# Autodesk Inventor assembly: 3.000 30A .500 With Adapters
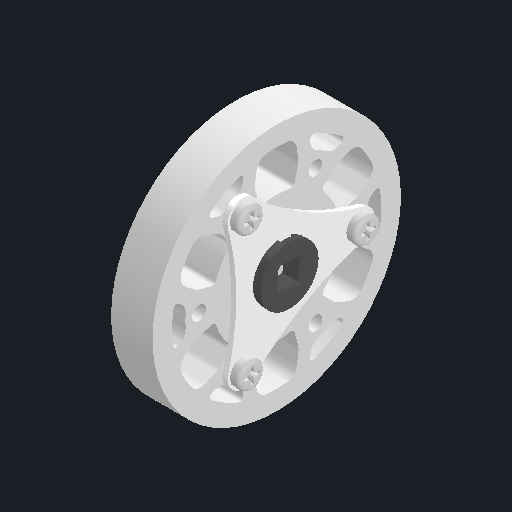
[picture p0: Inventor's stored thumbnail of the model, 512x512]
Saved by Autodesk Inventor 2025 (Build 290162000, 162)
## iProperties
Created: 2024-12-29
Part Number: 3.000 30A .500 With Adapters
Document SubType Name: Assembly
Designer: Averey Ku
Author: Averey Ku
## Documents named in this file (8)
- D:\VEX\High Stakes\CAD\ROBOPROS-CAD-Inventor\Quick Assemblies\3.000 30A .500 With Adapters.iam
- D:\VEX\High Stakes\CAD\ROBOPROS-CAD-Inventor\Motion\Wheels\Flex Wheels\3.000 Flex Wheel\3.000 30A .500.ipt
- D:\VEX\High Stakes\CAD\ROBOPROS-CAD-Inventor\Motion\Wheels\Flex Wheels\3.000 Flex Wheel.ipt
- D:\VEX\High Stakes\CAD\V4\Conveyer\Custom Parts\3 in Flex Wheel Hub.ipt
- D:\VEX\High Stakes\CAD\ROBOPROS-CAD-Inventor\Structure\Standoff\Standoff .50.ipt
- D:\VEX\High Stakes\CAD\ROBOPROS-CAD-Inventor\Structure\Standoff.ipt
- D:\VEX\High Stakes\CAD\ROBOPROS-CAD-Inventor\Structure\Hardware\Screw Nylon - Pan Head\NScrew Pan Head Threaded .250.ipt
- D:\VEX\High Stakes\CAD\ROBOPROS-CAD-Inventor\Motion\Wheels\Flex Wheels\VersaHex Adapters .125.ipt
## Components (14 placed, 5 different names)
1. 3.000 30A .500:1 — Flush:1, Mate:1, Mate:2, Insert:1, Mate:3, Insert:2, Mate:4, Insert:3, Mate:5, Mate:7
2. 3 in Flex Wheel Hub:1 — Insert:1, Mate:3, Insert:4, Insert:5, Insert:6, Insert:7, Insert:8, Insert:9, Mate:6
3. 3 in Flex Wheel Hub:2 — Insert:2, Mate:4, Insert:3, Insert:10, Insert:11, Insert:12, Mate:8
4. Standoff .50:1 — Insert:5
5. Standoff .50:2 — Insert:4
6. Standoff .50:3 — Insert:6
7. NScrew Pan Head Threaded .250:1 — Insert:7
8. NScrew Pan Head Threaded .250:2 — Insert:8
9. NScrew Pan Head Threaded .250:3 — Insert:9
10. NScrew Pan Head Threaded .250:4 — Insert:10
11. NScrew Pan Head Threaded .250:5 — Insert:11
12. NScrew Pan Head Threaded .250:6 — Insert:12
13. VersaHex Adapters .125:1 — Mate:7, Mate:8, Flush:2
14. VersaHex Adapters .125:2 — Mate:5, Mate:6, Flush:2
## Relationships (22: Insert 12, Mate 8, Flush 2)
- Flush:1 (-6.35 mm): 3.000 30A .500:1
- Mate:1: 3.000 30A .500:1
- Mate:2: 3.000 30A .500:1
- Insert:1: 3.000 30A .500:1 ↔ 3 in Flex Wheel Hub:1
- Mate:3: 3.000 30A .500:1 ↔ 3 in Flex Wheel Hub:1
- Insert:2: 3.000 30A .500:1 ↔ 3 in Flex Wheel Hub:2
- Mate:4: 3.000 30A .500:1 ↔ 3 in Flex Wheel Hub:2
- Insert:3: 3.000 30A .500:1 ↔ 3 in Flex Wheel Hub:2
- Insert:4: 3 in Flex Wheel Hub:1 ↔ Standoff .50:2
- Insert:5: 3 in Flex Wheel Hub:1 ↔ Standoff .50:1
- Insert:6: 3 in Flex Wheel Hub:1 ↔ Standoff .50:3
- Insert:7: 3 in Flex Wheel Hub:1 ↔ NScrew Pan Head Threaded .250:1
- Insert:8: 3 in Flex Wheel Hub:1 ↔ NScrew Pan Head Threaded .250:2
- Insert:9: 3 in Flex Wheel Hub:1 ↔ NScrew Pan Head Threaded .250:3
- Insert:10: 3 in Flex Wheel Hub:2 ↔ NScrew Pan Head Threaded .250:4
- Insert:11: 3 in Flex Wheel Hub:2 ↔ NScrew Pan Head Threaded .250:5
- Insert:12: 3 in Flex Wheel Hub:2 ↔ NScrew Pan Head Threaded .250:6
- Mate:5: 3.000 30A .500:1 ↔ VersaHex Adapters .125:2
- Mate:6: 3 in Flex Wheel Hub:1 ↔ VersaHex Adapters .125:2
- Mate:7: 3.000 30A .500:1 ↔ VersaHex Adapters .125:1
- Mate:8: 3 in Flex Wheel Hub:2 ↔ VersaHex Adapters .125:1
- Flush:2: VersaHex Adapters .125:1 ↔ VersaHex Adapters .125:2
